# Autodesk Inventor assembly: AK-C-C39-LED-Module
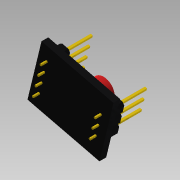
[picture p0: Inventor's stored thumbnail of the model, 180x180]
Saved by Autodesk Inventor 2016 (Build 200138000, 138)
## iProperties
Created: 2016-05-27
Part Number: AK-C-C39-LED-Module
Document SubType Name: Assembly
Designer: admin
Author: admin
## Documents named in this file (3)
- E:\Alex\DI-Lambda\parts\v1\AK-C-C39\AK-C-C39-LED-Module.iam
- E:\Alex\DI-Lambda\parts\v1\AK-C-C39\LED_module.ipt
- E:\Alex\DI-Lambda\parts\Common\Pin-round-2.54-male.ipt
## Components (8 placed, 2 different names)
1. LED_module:1 — Mate:6, Mate:7, Mate:8, Mate:9, Mate:10, Mate:11
2. Pin-round-2.54-male:1 — Flush:5, Flush:10, Mate:5, Mate:8
3. Pin-round-2.54-male:2 — Flush:4, Flush:5, Flush:9, Flush:10, Mate:4, Mate:5
4. Pin-round-2.54-male:3 — Flush:3, Flush:4, Flush:8, Flush:9, Mate:3, Mate:4, Mate:6
5. Pin-round-2.54-male:4 — Flush:3, Flush:8, Mate:3, Mate:9
6. Pin-round-2.54-male:5 — Flush:2, Flush:7, Mate:1, Mate:10
7. Pin-round-2.54-male:6 — Flush:1, Flush:2, Flush:6, Mate:2, Mate:11
8. Pin-round-2.54-male:7 — Flush:1, Flush:6, Flush:7, Mate:1, Mate:2, Mate:7
## Relationships (21: Mate 11, Flush 10)
- Flush:1: Pin-round-2.54-male:6 ↔ Pin-round-2.54-male:7
- Flush:2: Pin-round-2.54-male:5 ↔ Pin-round-2.54-male:6
- Flush:3: Pin-round-2.54-male:3 ↔ Pin-round-2.54-male:4
- Flush:4: Pin-round-2.54-male:2 ↔ Pin-round-2.54-male:3
- Flush:5: Pin-round-2.54-male:1 ↔ Pin-round-2.54-male:2
- Flush:6: Pin-round-2.54-male:6 ↔ Pin-round-2.54-male:7
- Flush:7: Pin-round-2.54-male:5 ↔ Pin-round-2.54-male:7
- Mate:1: Pin-round-2.54-male:5 ↔ Pin-round-2.54-male:7
- Mate:2: Pin-round-2.54-male:6 ↔ Pin-round-2.54-male:7
- Flush:8: Pin-round-2.54-male:3 ↔ Pin-round-2.54-male:4
- Flush:9: Pin-round-2.54-male:2 ↔ Pin-round-2.54-male:3
- Flush:10: Pin-round-2.54-male:1 ↔ Pin-round-2.54-male:2
- Mate:3: Pin-round-2.54-male:3 ↔ Pin-round-2.54-male:4
- Mate:4: Pin-round-2.54-male:2 ↔ Pin-round-2.54-male:3
- Mate:5: Pin-round-2.54-male:1 ↔ Pin-round-2.54-male:2
- Mate:6: LED_module:1 ↔ Pin-round-2.54-male:3
- Mate:7: LED_module:1 ↔ Pin-round-2.54-male:7
- Mate:8: LED_module:1 ↔ Pin-round-2.54-male:1
- Mate:9: LED_module:1 ↔ Pin-round-2.54-male:4
- Mate:10: LED_module:1 ↔ Pin-round-2.54-male:5
- Mate:11: LED_module:1 ↔ Pin-round-2.54-male:6
